# Autodesk Inventor assembly: Сборка2
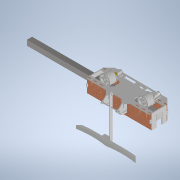
[picture p0: Inventor's stored thumbnail of the model, 180x180]
Saved by Autodesk Inventor 2020 (Build 240168000, 168)
## iProperties
Created: 2025-01-24
Part Number: Сборка2
Document SubType Name: Assembly
Designer: frozj
Author: frozj
## Documents named in this file (14)
- A:\frozjt\Documents\Модели\арканоид нью\Сборка2.iam
- A:\frozjt\Documents\Модели\арканоид нью\Деталь3.ipt
- A:\frozjt\Documents\Модели\арканоид нью\зад.ipt
- A:\frozjt\Documents\Модели\арканоид нью\перед.ipt
- A:\frozjt\Documents\Модели\арканоид нью\бок.ipt
- A:\frozjt\Documents\Модели\арканоид нью\дно.ipt
- A:\frozjt\Documents\Модели\арканоид нью\опора.ipt
- A:\frozjt\Documents\Модели\арканоид нью\крепление_мотора.ipt
- A:\frozjt\Documents\Модели\арканоид нью\Micro Metal Gear Motor.ipt
- A:\frozjt\Documents\Модели\арканоид\Wheel.ipt
- A:\frozjt\Documents\Модели\арканоид нью\балка.ipt
- A:\frozjt\Documents\Модели\арканоид нью\крепление оси.ipt
- D:\Модели\арканоид нью\ось_ударки.ipt
- D:\Модели\арканоид нью\пиналка_дер\Сборка_пиналка.iam
## Components (21 placed, 13 different names)
1. Деталь3:1 — С поворотом:1, Жесткий:1, С поворотом:9, С поворотом:10, С поворотом:12, С поворотом:13
2. зад:1 — С поворотом:1, С поворотом:3, С поворотом:8
3. перед:1 — Жесткий:1, С поворотом:2, С поворотом:4, С поворотом:5, С поворотом:6, Жесткий:2, Жесткий:3
4. бок:1 — С поворотом:2
5. дно:1 — С поворотом:3, С поворотом:7
6. бок:2 — С поворотом:4, С поворотом:15
7. опора:1 — С поворотом:5
8. опора:2 — С поворотом:6
9. опора:3 — С поворотом:7
10. опора:4 — С поворотом:8
11. крепление_мотора:1 — С поворотом:9
12. Micro Metal Gear Motor:1 — С поворотом:10, С поворотом:11
13. Wheel:1 — С поворотом:11
14. крепление_мотора:2 — С поворотом:12
15. Micro Metal Gear Motor:2 — С поворотом:13, С поворотом:14
16. Wheel:2 — С поворотом:14
17. балка:1 — С поворотом:15
18. крепление оси:1 — Жесткий:2, С поворотом:16
19. крепление оси:2 — Жесткий:3
20. ось_ударки:1 — С поворотом:16, С поворотом:17
21. Сборка_пиналка:1 [sub-assembly] — С поворотом:17
## Relationships (20: RevoluteJoint 17, WeldJoint 3)
- С поворотом:1 [RevoluteJoint]: Деталь3:1 ↔ зад:1
- Жесткий:1 [WeldJoint]: Деталь3:1 ↔ перед:1
- С поворотом:2 [RevoluteJoint]: перед:1 ↔ бок:1
- С поворотом:3 [RevoluteJoint]: зад:1 ↔ дно:1
- С поворотом:4 [RevoluteJoint]: перед:1 ↔ бок:2
- С поворотом:5 [RevoluteJoint]: перед:1 ↔ опора:1
- С поворотом:6 [RevoluteJoint]: перед:1 ↔ опора:2
- С поворотом:7 [RevoluteJoint]: дно:1 ↔ опора:3
- С поворотом:8 [RevoluteJoint]: зад:1 ↔ опора:4
- С поворотом:9 [RevoluteJoint]: Деталь3:1 ↔ крепление_мотора:1
- С поворотом:10 [RevoluteJoint]: Деталь3:1 ↔ Micro Metal Gear Motor:1
- С поворотом:11 [RevoluteJoint]: Micro Metal Gear Motor:1 ↔ Wheel:1
- С поворотом:12 [RevoluteJoint]: Деталь3:1 ↔ крепление_мотора:2
- С поворотом:13 [RevoluteJoint]: Деталь3:1 ↔ Micro Metal Gear Motor:2
- С поворотом:14 [RevoluteJoint]: Micro Metal Gear Motor:2 ↔ Wheel:2
- С поворотом:15 [RevoluteJoint]: бок:2 ↔ балка:1
- Жесткий:2 [WeldJoint]: перед:1 ↔ крепление оси:1
- Жесткий:3 [WeldJoint]: перед:1 ↔ крепление оси:2
- С поворотом:16 [RevoluteJoint]: крепление оси:1 ↔ ось_ударки:1
- С поворотом:17 [RevoluteJoint]: ось_ударки:1 ↔ Сборка_пиналка:1
